# Autodesk Inventor assembly: Jet Base Design
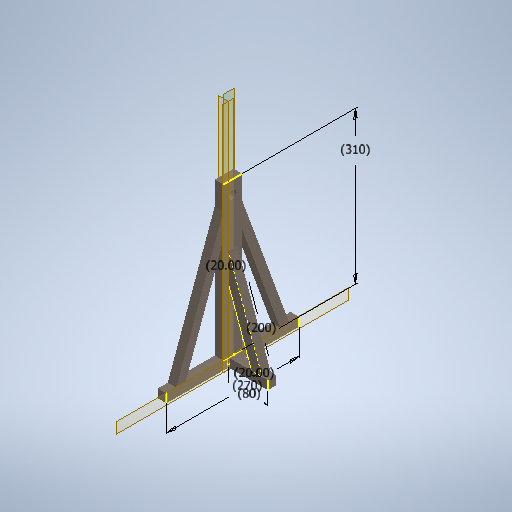
[picture p0: Inventor's stored thumbnail of the model, 512x512]
Saved by Autodesk Inventor 2025.2 (Build 292293000, 293)
## iProperties
Created: 2025-03-06
Part Number: Jet Base Design
Document SubType Name: Assembly
Designer: baolo
Author: baolo
## Documents named in this file (6)
- C:\Users\baolo\OneDrive\Desktop\the 2024 homework folder\engg 160\Trebuchet Models\Jet Base Design.iam
- C:\Users\baolo\OneDrive\Desktop\the 2024 homework folder\engg 160\Trebuchet Models\BaseLarge.ipt
- C:\Users\baolo\OneDrive\Desktop\the 2024 homework folder\engg 160\Trebuchet Models\BaseUpper.ipt
- C:\Users\baolo\OneDrive\Desktop\the 2024 homework folder\engg 160\Trebuchet Models\BaseAngularLarge.ipt
- C:\Users\baolo\OneDrive\Desktop\the 2024 homework folder\engg 160\Trebuchet Models\BaseSmall.ipt
- C:\Users\baolo\OneDrive\Desktop\the 2024 homework folder\engg 160\Trebuchet Models\BaseAngularSmall.ipt
## Components (6 placed, 5 different names)
1. BaseLarge:1 — Flush:1, Mate:1, Mate:2, Mate:3, Flush:2, Flush:3, Flush:4, Mate:4, Mate:7, Flush:9, Flush:10, Mate:8, Flush:11
2. BaseUpper:1 — Flush:1, Mate:1, Flush:2, Flush:3, Flush:5, Flush:6, Flush:7, Mate:5, Mate:6, Flush:8, Mate:10
3. BaseAngularLarge:1 — Flush:5, Flush:6, Flush:7, Mate:4, Mate:5
4. BaseAngularLarge:2 — Mate:6, Mate:7, Flush:8
5. BaseSmall:1 — Flush:9, Flush:10, Mate:8, Flush:11, Flush:15, Mate:9
6. BaseAngularSmall:1 — Flush:15, Mate:9, Mate:10
## Relationships (22: Flush 12, Mate 10)
- Flush:1: BaseLarge:1 ↔ BaseUpper:1
- Mate:1: BaseLarge:1 ↔ BaseUpper:1
- Mate:2: BaseLarge:1
- Mate:3 (20 mm): BaseLarge:1
- Flush:2: BaseLarge:1 ↔ BaseUpper:1
- Flush:3: BaseLarge:1 ↔ BaseUpper:1
- Flush:4: BaseLarge:1
- Flush:5: BaseUpper:1 ↔ BaseAngularLarge:1
- Flush:6: BaseUpper:1 ↔ BaseAngularLarge:1
- Flush:7: BaseUpper:1 ↔ BaseAngularLarge:1
- Mate:4: BaseLarge:1 ↔ BaseAngularLarge:1
- Mate:5: BaseUpper:1 ↔ BaseAngularLarge:1
- Mate:6: BaseUpper:1 ↔ BaseAngularLarge:2
- Mate:7: BaseLarge:1 ↔ BaseAngularLarge:2
- Flush:8: BaseUpper:1 ↔ BaseAngularLarge:2
- Flush:9: BaseLarge:1 ↔ BaseSmall:1
- Flush:10: BaseLarge:1 ↔ BaseSmall:1
- Mate:8: BaseLarge:1 ↔ BaseSmall:1
- Flush:11: BaseLarge:1 ↔ BaseSmall:1
- Flush:15: BaseSmall:1 ↔ BaseAngularSmall:1
- Mate:9: BaseSmall:1 ↔ BaseAngularSmall:1
- Mate:10: BaseUpper:1 ↔ BaseAngularSmall:1
